# Autodesk Inventor assembly: nucleoWithShield
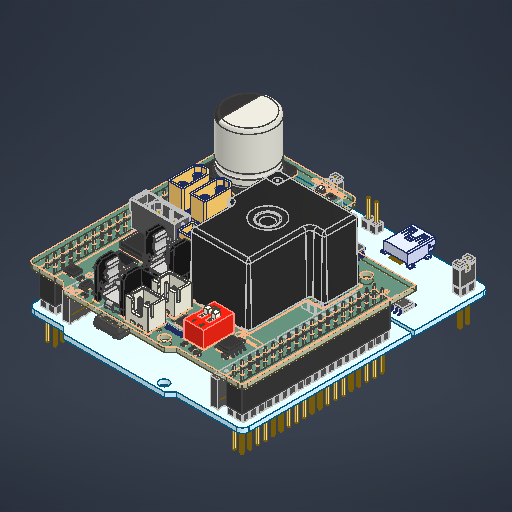
[picture p0: Inventor's stored thumbnail of the model, 512x512]
Saved by Autodesk Inventor 2026 (Build 300175050, 175E)
## iProperties
Created: 2026-05-22
Part Number: nucleoWithShield
Document SubType Name: Assembly
Designer: anawa
Author: anawa
## Documents named in this file (3)
- D:\Nano\Another_Job\AjYui_motor_brake\MotorBrake_shield\3D\nucleoWithShield.iam
- D:\Nano\Another_Job\AjYui_motor_brake\MotorBrake_shield\PCB\PCB\PCB.ipt
- D:\Nano\Another_Job\AjYui_motor_brake\MotorBrake_shield\3D\NUCLEO-F446RE--3DModel-STEP-56544\NUCLEO-F446RE--3DModel-STEP-56544\NUCLEO-F446RE--3DModel-STEP-56544.ipt
## Components (2 placed, 2 different names)
1. PCB:1 — Flush:1, Flush:2, Mate:1
2. NUCLEO-F446RE--3DModel-STEP-56544:1 — Flush:1, Flush:2, Mate:1
## Relationships (3: Flush 2, Mate 1)
- Flush:1: PCB:1 ↔ NUCLEO-F446RE--3DModel-STEP-56544:1
- Flush:2: PCB:1 ↔ NUCLEO-F446RE--3DModel-STEP-56544:1
- Mate:1: PCB:1 ↔ NUCLEO-F446RE--3DModel-STEP-56544:1
